# Autodesk Inventor assembly: DCmotor40W
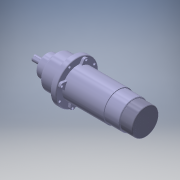
[picture p0: Inventor's stored thumbnail of the model, 180x180]
Saved by Autodesk Inventor 2018 (Build 220112000, 112)
## iProperties
Created: 2017-09-12
Part Number: DCmotor40W
Material: 一般
Document SubType Name: Assembly
Designer: 翔
Source: UnKnown
Author: 翔
## Documents named in this file (4)
- E:\forest_robot_cad\Forest_v4\wheel\DCmotor40W.iam
- E:\forest_robot_cad\Forest_v4\wheel\Motor40W.ipt
- E:\forest_robot_cad\Forest_v4\wheel\ShaftDC40W.ipt
- E:\forest_robot_cad\Forest_v4\wheel\Encoder_4e2-e.ipt
## Components (3 placed, 3 different names)
1. Motor40W.1 — メイト:1, メイト:2
2. ShaftDC40W.1 — メイト:1, メイト:2
3. Encoder_4e2-e.1
## Relationships (2: Mate 2)
- メイト:1 [Mate]: Motor40W.1 ↔ ShaftDC40W.1
- メイト:2 [Mate]: Motor40W.1 ↔ ShaftDC40W.1
